# Autodesk Inventor assembly: Assembly_v2
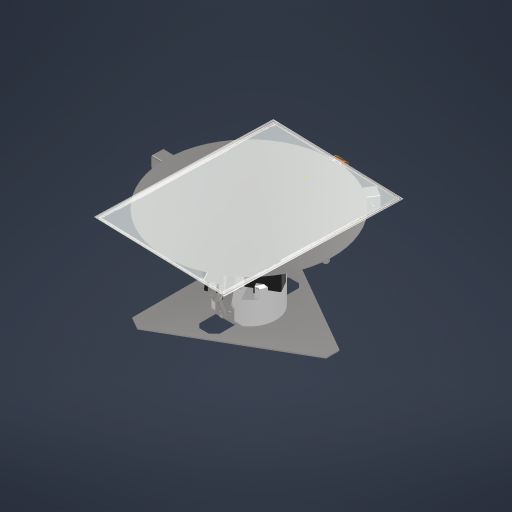
[picture p0: Inventor's stored thumbnail of the model, 512x512]
Saved by Autodesk Inventor 2023 (Build 270158000, 158)
## iProperties
Created: 2023-02-25
Part Number: Assembly_v2
Document SubType Name: Assembly
Designer: roota
Mass: 2505.51 g
Surface Area: 3613.46 cm^2
Volume: 474.073 cm^3
Density: 5.28507 g/cm^3
Author: roota
## Documents named in this file (21)
- D:\GitHub\NTUST-Mechanical-Design\Ball stabilization mechanism\3D CAD files\Mechanical Part CAD files\Assemblies\Assembly_v2.iam
- D:\GitHub\NTUST-Mechanical-Design\Ball stabilization mechanism\3D CAD files\Mechanical Part CAD files\Static Mechanisms\BalancePlate.ipt
- D:\GitHub\NTUST-Mechanical-Design\Ball stabilization mechanism\3D CAD files\Mechanical Part CAD files\Static Mechanisms\BasePlate.ipt
- D:\GitHub\NTUST-Mechanical-Design\Ball stabilization mechanism\3D CAD files\Mechanical Part CAD files\Static Mechanisms\BaseSupport.ipt
- D:\GitHub\NTUST-Mechanical-Design\Ball stabilization mechanism\3D CAD files\Electrical Hardware CAD files\SERVO\LDX-335MG_Servo_15kg_cm.ipt
- C:\Users\roota\Documents\Inventor\Content Center Files\R2023\en-US\ISO 10642(1)\ISO 10642 - M8 x  60.ipt
- C:\Users\roota\Documents\Inventor\Content Center Files\R2023\en-US\ISO 4762(2)\ISO 4762 - M5 x 8ISO.ipt
- C:\Users\roota\Documents\Inventor\Content Center Files\R2023\en-US\ISO 4026\ISO 4026 - M3 x 6 - ISO.ipt
- D:\GitHub\NTUST-Mechanical-Design\Ball stabilization mechanism\3D CAD files\Mechanical Part CAD files\Hardware Parts\5mm Bushing.ipt
- D:\GitHub\NTUST-Mechanical-Design\Ball stabilization mechanism\3D CAD files\Mechanical Part CAD files\Hardware Parts\M6x1_THREADED_ROD.ipt
- D:\GitHub\NTUST-Mechanical-Design\Ball stabilization mechanism\3D CAD files\Mechanical Part CAD files\Hardware Parts\SELF-LUBRIFICATING ROD END\End_6mm.ipt
- D:\GitHub\NTUST-Mechanical-Design\Ball stabilization mechanism\3D CAD files\Mechanical Part CAD files\Hardware Parts\SELF-LUBRIFICATING ROD END\Ball_6mm.ipt
- D:\GitHub\NTUST-Mechanical-Design\Ball stabilization mechanism\3D CAD files\Mechanical Part CAD files\Static Mechanisms\4mm spacer.ipt
- D:\GitHub\NTUST-Mechanical-Design\Ball stabilization mechanism\3D CAD files\Mechanical Part CAD files\Static Mechanisms\rod pin.ipt
- C:\Users\roota\Documents\Inventor\Content Center Files\R2023\en-US\JIS B 2804 E\_JIS B 2804 E - 5 - 6.ipt
- C:\Users\roota\Documents\Inventor\Content Center Files\R2023\en-US\ISO 4036(2)\ISO 4036 - M6(2).ipt
- D:\GitHub\NTUST-Mechanical-Design\Ball stabilization mechanism\3D CAD files\Mechanical Part CAD files\Hardware Parts\12_1_INCH_TOUCHSCREEN\12inch Touchscreen.ipt
- D:\GitHub\NTUST-Mechanical-Design\Ball stabilization mechanism\3D CAD files\Mechanical Part CAD files\Dynamic Mechanisms\Servo_Strut_v2.ipt
- D:\GitHub\NTUST-Mechanical-Design\Ball stabilization mechanism\3D CAD files\Electrical Hardware CAD files\ARDUINO_UNO\Arduino_Uno.ipt
- D:\GitHub\NTUST-Mechanical-Design\Ball stabilization mechanism\3D CAD files\Mechanical Part CAD files\Static Mechanisms\ServoCap V2.ipt
- C:\Users\roota\Documents\Inventor\Content Center Files\R2023\en-US\ISO 4762(2)\ISO 4762 - M3 x 8ISO.ipt
## Components (59 placed, 20 different names)
1. BalancePlate:1 — Mate:19, Mate:20, Mate:21, Mate:22, Mate:23, Mate:24, Mate:26, Mate:28, Mate:30, Mate:31, Flush:1, Flush:2, Mate:44
2. BasePlate:1 — Mate:1, Mate:2, Mate:3, Insert:13, Insert:14, Insert:15, Insert:16, Angle:4, Angle:5, Mate:45, Angle:6, Mate:46, Mate:47, Mate:48
3. BaseSupport:1 — Mate:1, Mate:2, Mate:3, Mate:4, Mate:5, Mate:6, Mate:7, Mate:8, Mate:9, Mate:10, Mate:11, Mate:12, Mate:17, Mate:18, Insert:17, Mate:44, Flush:3, Flush:4, Mate:49
4. LDX-335MG_Servo_15kg_cm:1 — Mate:4, Mate:7, Mate:10, Insert:49, Insert:55, Insert:56
5. LDX-335MG_Servo_15kg_cm:2 — Mate:5, Mate:8, Mate:11, Insert:50, Insert:53, Insert:54
6. LDX-335MG_Servo_15kg_cm:3 — Mate:6, Mate:9, Mate:12, Insert:48, Mate:51, Mate:53, Insert:51, Insert:52
7. ISO 10642 M8x60:1 — Mate:49, Mate:50, Mate:52
8. ISO 4762 M5 x 8:13 — Insert:13
9. ISO 4762 M5 x 8:14 — Insert:14
10. ISO 4762 M5 x 8:15 — Insert:15
11. ISO 4762 M5 x 8:16 — Insert:16
12. ISO 4026 M3 x 6:1 — Mate:17, Flush:4
13. ISO 4026 M3 x 6:2 — Mate:18, Flush:3
14. ISO 4026 M3 x 6:3 — Insert:17
15. 5mm Bushing:1 — Mate:36, Mate:38, Mate:54
16. 5mm Bushing:2 — Mate:32, Mate:33, Mate:34
17. 5mm Bushing:3 — Mate:39, Mate:40, Insert:57
18. M6x1_THREADED_ROD:1 — Insert:32, Angle:3, Mate:34, Mate:35
19. M6x1_THREADED_ROD:2 — Insert:31, Angle:2, Mate:36, Mate:43
20. M6x1_THREADED_ROD:3 — Insert:30, Angle:1, Mate:39, Mate:41
21. End_6mm:1 — Insert:30, Tangent:2, Angle:1, Insert:46
22. End_6mm:2 — Insert:31, Tangent:3, Angle:2, Insert:47
23. End_6mm:3 — Insert:32, Tangent:1, Angle:3, Insert:45
24. Ball_6mm:1 — Tangent:1, Insert:34, Insert:35
25. Ball_6mm:2 — Tangent:2, Insert:36, Insert:37
26. Ball_6mm:3 — Tangent:3, Insert:33, Insert:38
27. 4mm spacer:1 — Insert:33
28. 4mm spacer:3 — Insert:34
29. 4mm spacer:4 — Insert:35, Mate:27, Mate:28
30. 4mm spacer:5 — Insert:36
31. 4mm spacer:6 — Insert:37, Mate:29, Mate:30
32. 4mm spacer:7 — Insert:38, Mate:25, Mate:26
33. rod pin:1 — Insert:39, Insert:40, Mate:19, Mate:27
34. rod pin:2 — Insert:41, Insert:42, Mate:20, Mate:25
35. rod pin:3 — Insert:43, Insert:44, Mate:21, Mate:29
36. JIS B 2804 E 5:1 — Insert:39
37. JIS B 2804 E 5:2 — Insert:40, Mate:22
38. JIS B 2804 E 5:3 — Insert:41, Mate:23
39. JIS B 2804 E 5:4 — Insert:42
40. JIS B 2804 E 5:5 — Insert:43, Mate:24
41. JIS B 2804 E 5:6 — Insert:44
42. ISO 4036 M6:1 — Insert:45
43. ISO 4036 M6:2 — Insert:46
44. ISO 4036 M6:3 — Insert:47
45. 12inch Touchscreen:1 — Mate:31, Flush:1, Flush:2, Angle:4, Angle:5
46. Servo_Strut_v2:1 — Insert:48, Mate:38, Mate:43, Mate:55, Mate:56
47. Servo_Strut_v2:2 — Insert:49, Mate:40, Mate:41, Mate:57
48. Servo_Strut_v2:3 — Insert:50, Mate:32, Mate:33, Mate:35, Insert:58
49. Arduino_Uno:1 — Mate:45, Angle:6
50. ServoCap V2:1 — Mate:50, Mate:51, Mate:52, Mate:53
51. ISO 4762 M5 x 8:17 — Insert:51
52. ISO 4762 M5 x 8:18 — Insert:52
53. ISO 4762 M5 x 8:19 — Insert:53
54. ISO 4762 M5 x 8:20 — Insert:54
55. ISO 4762 M5 x 8:21 — Insert:55
56. ISO 4762 M5 x 8:22 — Insert:56
57. ISO 4762 M3 x 8:1 — Insert:57, Mate:57
58. ISO 4762 M3 x 8:2 — Mate:54, Mate:55, Mate:56
59. ISO 4762 M3 x 8:3 — Insert:58
## Relationships (98: Mate 51, Insert 34, Angle 6, Flush 4, Tangent 3)
- Mate:1: BasePlate:1 ↔ BaseSupport:1
- Mate:2: BasePlate:1 ↔ BaseSupport:1
- Mate:3: BasePlate:1 ↔ BaseSupport:1
- Mate:4: BaseSupport:1 ↔ LDX-335MG_Servo_15kg_cm:1
- Mate:5: BaseSupport:1 ↔ LDX-335MG_Servo_15kg_cm:2
- Mate:6: BaseSupport:1 ↔ LDX-335MG_Servo_15kg_cm:3
- Mate:7: BaseSupport:1 ↔ LDX-335MG_Servo_15kg_cm:1
- Mate:8: BaseSupport:1 ↔ LDX-335MG_Servo_15kg_cm:2
- Mate:9: BaseSupport:1 ↔ LDX-335MG_Servo_15kg_cm:3
- Mate:10: BaseSupport:1 ↔ LDX-335MG_Servo_15kg_cm:1
- Mate:11: BaseSupport:1 ↔ LDX-335MG_Servo_15kg_cm:2
- Mate:12: BaseSupport:1 ↔ LDX-335MG_Servo_15kg_cm:3
- Insert:13: BasePlate:1 ↔ ISO 4762 M5 x 8:13
- Insert:14: BasePlate:1 ↔ ISO 4762 M5 x 8:14
- Insert:15: BasePlate:1 ↔ ISO 4762 M5 x 8:15
- Insert:16: BasePlate:1 ↔ ISO 4762 M5 x 8:16
- Mate:17: BaseSupport:1 ↔ ISO 4026 M3 x 6:1
- Mate:18: BaseSupport:1 ↔ ISO 4026 M3 x 6:2
- Insert:17: BaseSupport:1 ↔ ISO 4026 M3 x 6:3
- Insert:30 (-10 mm): M6x1_THREADED_ROD:3 ↔ End_6mm:1
- Insert:31 (-10 mm): M6x1_THREADED_ROD:2 ↔ End_6mm:2
- Insert:32 (-10 mm): M6x1_THREADED_ROD:1 ↔ End_6mm:3
- Tangent:1: End_6mm:3 ↔ Ball_6mm:1
- Tangent:2: End_6mm:1 ↔ Ball_6mm:2
- Tangent:3: End_6mm:2 ↔ Ball_6mm:3
- Insert:33: Ball_6mm:3 ↔ 4mm spacer:1
- Insert:34: Ball_6mm:1 ↔ 4mm spacer:3
- Insert:35: Ball_6mm:1 ↔ 4mm spacer:4
- Insert:36: Ball_6mm:2 ↔ 4mm spacer:5
- Insert:37: Ball_6mm:2 ↔ 4mm spacer:6
- Insert:38: Ball_6mm:3 ↔ 4mm spacer:7
- Insert:39: rod pin:1 ↔ JIS B 2804 E 5:1
- Insert:40: rod pin:1 ↔ JIS B 2804 E 5:2
- Insert:41: rod pin:2 ↔ JIS B 2804 E 5:3
- Insert:42: rod pin:2 ↔ JIS B 2804 E 5:4
- Insert:43: rod pin:3 ↔ JIS B 2804 E 5:5
- Insert:44: rod pin:3 ↔ JIS B 2804 E 5:6
- Mate:19: BalancePlate:1 ↔ rod pin:1
- Mate:20: BalancePlate:1 ↔ rod pin:2
- Mate:21: BalancePlate:1 ↔ rod pin:3
- Mate:22: BalancePlate:1 ↔ JIS B 2804 E 5:2
- Mate:23: BalancePlate:1 ↔ JIS B 2804 E 5:3
- Mate:24: BalancePlate:1 ↔ JIS B 2804 E 5:5
- Mate:25: 4mm spacer:7 ↔ rod pin:2
- Mate:26: BalancePlate:1 ↔ 4mm spacer:7
- Mate:27: 4mm spacer:4 ↔ rod pin:1
- Mate:28: BalancePlate:1 ↔ 4mm spacer:4
- Mate:29: 4mm spacer:6 ↔ rod pin:3
- Mate:30: BalancePlate:1 ↔ 4mm spacer:6
- Angle:1 (0 deg): M6x1_THREADED_ROD:3 ↔ End_6mm:1
- Angle:2 (0 deg): M6x1_THREADED_ROD:2 ↔ End_6mm:2
- Angle:3 (0 deg): M6x1_THREADED_ROD:1 ↔ End_6mm:3
- Insert:45: End_6mm:3 ↔ ISO 4036 M6:1
- Insert:46: End_6mm:1 ↔ ISO 4036 M6:2
- Insert:47: End_6mm:2 ↔ ISO 4036 M6:3
- Mate:31: BalancePlate:1 ↔ 12inch Touchscreen:1
- Flush:1 (-120 mm): BalancePlate:1 ↔ 12inch Touchscreen:1
- Flush:2 (40 mm): BalancePlate:1 ↔ 12inch Touchscreen:1
- Insert:48: LDX-335MG_Servo_15kg_cm:3 ↔ Servo_Strut_v2:1
- Insert:49: LDX-335MG_Servo_15kg_cm:1 ↔ Servo_Strut_v2:2
- Insert:50: LDX-335MG_Servo_15kg_cm:2 ↔ Servo_Strut_v2:3
- Mate:32: 5mm Bushing:2 ↔ Servo_Strut_v2:3
- Mate:33: 5mm Bushing:2 ↔ Servo_Strut_v2:3
- Mate:34: 5mm Bushing:2 ↔ M6x1_THREADED_ROD:1
- Mate:35: M6x1_THREADED_ROD:1 ↔ Servo_Strut_v2:3
- Mate:36: 5mm Bushing:1 ↔ M6x1_THREADED_ROD:2
- Mate:38: 5mm Bushing:1 ↔ Servo_Strut_v2:1
- Mate:39: 5mm Bushing:3 ↔ M6x1_THREADED_ROD:3
- Mate:40: 5mm Bushing:3 ↔ Servo_Strut_v2:2
- Mate:41: M6x1_THREADED_ROD:3 ↔ Servo_Strut_v2:2
- Mate:43: M6x1_THREADED_ROD:2 ↔ Servo_Strut_v2:1
- Angle:4 (90 deg): BasePlate:1 ↔ 12inch Touchscreen:1
- Angle:5 (-90 deg): BasePlate:1 ↔ 12inch Touchscreen:1
- Mate:44 (90 mm): BalancePlate:1 ↔ BaseSupport:1
- Mate:45: BasePlate:1 ↔ Arduino_Uno:1
- Angle:6 (0 deg): BasePlate:1 ↔ Arduino_Uno:1
- Mate:46: BasePlate:1
- Mate:47: BasePlate:1
- Mate:48: BasePlate:1
- Flush:3: BaseSupport:1 ↔ ISO 4026 M3 x 6:2
- Flush:4: BaseSupport:1 ↔ ISO 4026 M3 x 6:1
- Mate:49: BaseSupport:1 ↔ ISO 10642 M8x60:1
- Mate:50: ISO 10642 M8x60:1 ↔ ServoCap V2:1
- Mate:51: LDX-335MG_Servo_15kg_cm:3 ↔ ServoCap V2:1
- Mate:52: ISO 10642 M8x60:1 ↔ ServoCap V2:1
- Mate:53: LDX-335MG_Servo_15kg_cm:3 ↔ ServoCap V2:1
- Insert:51: LDX-335MG_Servo_15kg_cm:3 ↔ ISO 4762 M5 x 8:17
- Insert:52: LDX-335MG_Servo_15kg_cm:3 ↔ ISO 4762 M5 x 8:18
- Insert:53: LDX-335MG_Servo_15kg_cm:2 ↔ ISO 4762 M5 x 8:19
- Insert:54: LDX-335MG_Servo_15kg_cm:2 ↔ ISO 4762 M5 x 8:20
- Insert:55: LDX-335MG_Servo_15kg_cm:1 ↔ ISO 4762 M5 x 8:21
- Insert:56: LDX-335MG_Servo_15kg_cm:1 ↔ ISO 4762 M5 x 8:22
- Insert:57: 5mm Bushing:3 ↔ ISO 4762 M3 x 8:1
- Insert:58: Servo_Strut_v2:3 ↔ ISO 4762 M3 x 8:3
- Mate:54: 5mm Bushing:1 ↔ ISO 4762 M3 x 8:2
- Mate:55: Servo_Strut_v2:1 ↔ ISO 4762 M3 x 8:2
- Mate:56: Servo_Strut_v2:1 ↔ ISO 4762 M3 x 8:2
- Mate:57: Servo_Strut_v2:2 ↔ ISO 4762 M3 x 8:1
## Named parameters: AngleX = 0 deg, AngleY = 0 deg
